# Autodesk Inventor assembly: Cuartof
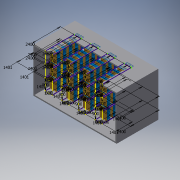
[picture p0: Inventor's stored thumbnail of the model, 180x180]
Saved by Autodesk Inventor 2016 (Build 200138000, 138)
## iProperties
Created: 2015-11-12
Part Number: Cuartof
Document SubType Name: Assembly
Designer: serge
Mass: 1.06776e+07 g
Surface Area: 3.91453e+06 cm^2
Volume: 1.06776e+07 cm^3
Density: 1 g/cm^3
Author: serge
## Documents named in this file (8)
- D:\Programas\xampp\htdocs\localUnal\storage\macros\cuarto\Modelado\Cuartof.iam
- D:\Programas\xampp\htdocs\localUnal\storage\macros\cuarto\Modelado\Cuarto\Cuarto.iam
- D:\Programas\xampp\htdocs\localUnal\storage\macros\cuarto\Modelado\Unidades\Evaporadora.ipt
- D:\Programas\xampp\htdocs\localUnal\storage\macros\cuarto\Modelado\estanteria.iam
- D:\Programas\xampp\htdocs\localUnal\storage\macros\cuarto\Modelado\Unidades\Condensadora.ipt
- D:\Programas\xampp\htdocs\localUnal\storage\macros\cuarto\Modelado\Soporte Unidades\Soporte.iam
- D:\Programas\xampp\htdocs\localUnal\storage\macros\cuarto\Modelado\Soporte Unidades\Soporte2.iam
- D:\Programas\xampp\htdocs\localUnal\storage\macros\cuarto\Modelado\Puente inventor.xlsx
## Components (8 placed, 6 different names)
1. Cuarto:1 [sub-assembly] — Flush:1, Mate:1, Mate:2, Coincidencia:3, Coincidencia:4, Nivelación:2, Coincidencia:5, Nivelación:3, Nivelación:4, Coincidencia:6, Coincidencia:9
2. Evaporadora:1 — Flush:1, Mate:1, Mate:2, Coincidencia:7, Nivelación:7, Nivelación:8
3. estanteria:1 [sub-assembly] — Coincidencia:3, Coincidencia:4, Nivelación:2
4. Condensadora:1 — Coincidencia:5, Nivelación:3, Nivelación:4, Coincidencia:8, Nivelación:11, Nivelación:12
5. Soporte:1 [sub-assembly] — Nivelación:5, Nivelación:6, Coincidencia:6, Coincidencia:7, Nivelación:8
6. Soporte:2 [sub-assembly] — Nivelación:5, Nivelación:6, Nivelación:7
7. Soporte2:1 [sub-assembly] — Nivelación:9, Nivelación:10, Coincidencia:8, Nivelación:12
8. Soporte2:2 [sub-assembly] — Nivelación:9, Nivelación:10, Nivelación:11, Coincidencia:9
## Relationships (21: Flush 12, Mate 9)
- Flush:1 (85 mm): Cuarto:1 ↔ Evaporadora:1
- Mate:1 (20 mm): Cuarto:1 ↔ Evaporadora:1
- Mate:2 (2164.5 mm): Cuarto:1 ↔ Evaporadora:1
- Coincidencia:3 [Mate] (1100 mm): Cuarto:1 ↔ estanteria:1
- Coincidencia:4 [Mate] (749 mm): Cuarto:1 ↔ estanteria:1
- Nivelación:2 [Flush]: Cuarto:1 ↔ estanteria:1
- Coincidencia:5 [Mate] (20 mm): Cuarto:1 ↔ Condensadora:1
- Nivelación:3 [Flush] (2842.775 mm): Cuarto:1 ↔ Condensadora:1
- Nivelación:4 [Flush] (35 mm): Cuarto:1 ↔ Condensadora:1
- Nivelación:5 [Flush]: Soporte:1 ↔ Soporte:2
- Nivelación:6 [Flush]: Soporte:1 ↔ Soporte:2
- Coincidencia:6 [Mate]: Cuarto:1 ↔ Soporte:1
- Coincidencia:7 [Mate]: Evaporadora:1 ↔ Soporte:1
- Nivelación:7 [Flush] (30 mm): Evaporadora:1 ↔ Soporte:2
- Nivelación:8 [Flush] (30 mm): Evaporadora:1 ↔ Soporte:1
- Nivelación:9 [Flush]: Soporte2:1 ↔ Soporte2:2
- Nivelación:10 [Flush]: Soporte2:1 ↔ Soporte2:2
- Coincidencia:8 [Mate]: Condensadora:1 ↔ Soporte2:1
- Nivelación:11 [Flush] (30 mm): Condensadora:1 ↔ Soporte2:2
- Nivelación:12 [Flush] (30 mm): Condensadora:1 ↔ Soporte2:1
- Coincidencia:9 [Mate]: Cuarto:1 ↔ Soporte2:2
## Named parameters: AET = 85 mm, EEP = 20 mm, A_ET = 35 mm, E_EP = 20 mm, PL_N = 7000 mm, PA_N = 3500 mm, PE_N = 101.6 mm, PL_S = 7000 mm, PA_S = 3500 mm, PE_S = 101.6 mm, DP_S = 4250 mm, AP_S = 2000 mm, PL_EO = 3500 mm, PA_EO = 3500 mm, PE_EO = 101.6 mm, T_L = 7000 mm, T_A = 3500 mm, T_E = 101.6 mm, lon_ve = 512.5 mm, n_a = 3 mm, t_a = 19.05 mm, d_a = 128.125 mm, lon_ho = 749 mm, d_bor = 59.92 mm, lon_gui = 187.25 mm, esp_gui = 461.25 mm, lon_ve2 = 498.475 mm, n_a2 = 3 mm, t_a2 = 124.61875 mm, d_a2 = 124.61875 mm, lon_ho2 = 933.45 mm, d_bor2 = 74.676 mm, lon_gui2 = 233.3625 mm, esp_gui2 = 448.6275 mm, UE_L = 2671 mm, UE_A = 1025 mm, UE_AN = 749 mm, UC_L = 1314.45 mm, UC_A = 996.95 mm, UC_AN = 933.45 mm, SEP_NS = 0 mm, SEP_EW = 1400 mm, CEP_NS = 1, CEP_EW = 4, DSEG = 0 mm, AEGEP_NS = 0 mm, SEPEG_NS = 100 mm, SEG_NS = 1000 mm, SEG_EW = 1400 mm, CEG_NS = 2, CEG_EW = 4, DNS = 749 mm, DEW = 1100 mm, DISTANCIAPAREDESTE = 1100 mm, DISTANCIAPAREDNORTE = 749 mm, ECP = 20 mm, EAP = 2842.775 mm, ACT = 35 mm
